# Autodesk Inventor assembly: GRIPPERFINAL51
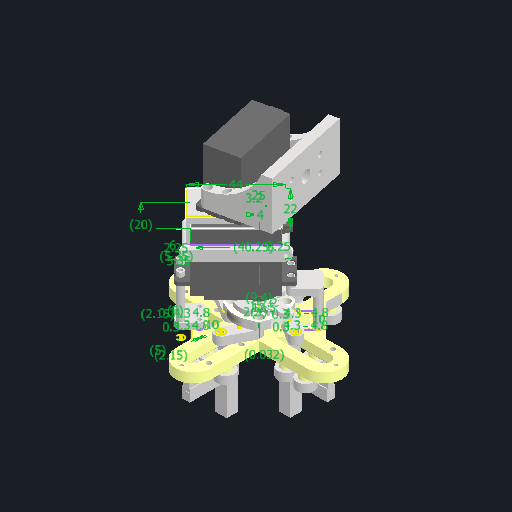
[picture p0: Inventor's stored thumbnail of the model, 512x512]
Saved by Autodesk Inventor 2026 (Build 300175000, 175)
## iProperties
Created: 2025-05-01
Part Number: GRIPPERFINAL51
Document SubType Name: Assembly
Designer: m_kni
Author: m_kni
## Documents named in this file (11)
- C:\Users\jerem\Documents\GitHub\Perovskite-Automated-Synthesis-System\CAD\Gripper\GRIPPERFINAL51.iam
- C:\Users\jerem\Documents\GitHub\Perovskite-Automated-Synthesis-System\CAD\Gripper\ALUMFINGER.ipt
- C:\Users\jerem\Documents\GitHub\Perovskite-Automated-Synthesis-System\CAD\Gripper\Assembly1.iam
- C:\Users\jerem\Documents\GitHub\Perovskite-Automated-Synthesis-System\CAD\Gripper\servostrap.ipt
- C:\Users\jerem\Documents\GitHub\Perovskite-Automated-Synthesis-System\CAD\Gripper\UpperGripperfingerpart.ipt
- C:\Users\jerem\Documents\GitHub\Perovskite-Automated-Synthesis-System\CAD\Non 3D Printed Parts\Bearings\5x5x11bearing.ipt
- C:\Users\jerem\Documents\GitHub\Perovskite-Automated-Synthesis-System\CAD\Gripper\Redesign_Linkage.ipt
- C:\Users\jerem\Documents\GitHub\Perovskite-Automated-Synthesis-System\CAD\Gripper\3x5x5bushing.ipt
- C:\Users\jerem\Documents\GitHub\Perovskite-Automated-Synthesis-System\CAD\Non 3D Printed Parts\Motors and Servos\MG 996R.ipt
- C:\Users\jerem\Documents\GitHub\Perovskite-Automated-Synthesis-System\CAD\Non 3D Printed Parts\Motors and Servos\MG996 2 Arm Pad.ipt
- C:\Users\jerem\Documents\GitHub\Perovskite-Automated-Synthesis-System\CAD\Gripper\SERVO_TO_TOOLHEAD.ipt
## Components (33 placed, 10 different names)
1. ALUMFINGER:1 — Insert:26, Angle:1
2. Assembly1:1 [sub-assembly] — Insert:1, Insert:2, Insert:3, Insert:4, Insert:5, Insert:6, Insert:7, Insert:8, Insert:9, Insert:10, Insert:11, Insert:12, Insert:13, Mate:8, Angle:5, Mate:13
3. servostrap:1 — Insert:1
4. UpperGripperfingerpart:1 — Mate:5, Tangent:3, Mate:6, Insert:29, Angle:4
5. UpperGripperfingerpart:2 — Mate:6, Tangent:4, Mate:7, Insert:27, Angle:2
6. UpperGripperfingerpart:3 — Tangent:1, Mate:1, Mate:2, Insert:28, Angle:3
7. UpperGripperfingerpart:4 — Mate:2, Tangent:2, Mate:3, Insert:26, Angle:1
8. 5x5x11bearing:1 — Insert:7
9. 5x5x11bearing:2 — Insert:6
10. 5x5x11bearing:3 — Insert:5, Tangent:1, Mate:1
11. 5x5x11bearing:4 — Insert:3, Mate:5
12. 5x5x11bearing:5 — Insert:2
13. 5x5x11bearing:6 — Insert:4, Tangent:3
14. 5x5x11bearing:7 — Insert:10, Tangent:2
15. 5x5x11bearing:8 — Insert:8
16. 5x5x11bearing:9 — Insert:11, Tangent:4, Mate:7
17. 5x5x11bearing:10 — Insert:9, Mate:3
18. 5x5x11bearing:11 — Insert:12
19. 5x5x11bearing:12 — Insert:13
20. Redesign_Linkage:1 — Insert:15
21. Redesign_Linkage:2 — Insert:24
22. Redesign_Linkage:3 — Insert:22
23. Redesign_Linkage:4 — Insert:20
24. 3x5x5bushing:5 — Insert:15
25. 3x5x5bushing:6 — Insert:22
26. 3x5x5bushing:7 — Insert:24
27. 3x5x5bushing:8 — Insert:20
28. ALUMFINGER:2 — Insert:27, Angle:2
29. ALUMFINGER:3 — Insert:28, Angle:3
30. ALUMFINGER:4 — Insert:29, Angle:4
31. MG 996R:1 — Mate:9, Mate:10, Mate:11, Mate:12, Angle:6
32. MG996 2 Arm Pad:1 — Mate:8, Angle:5, Mate:9, Mate:10, Mate:13
33. SERVO_TO_TOOLHEAD:1 — Mate:11, Mate:12, Angle:6
## Relationships (43: Insert 21, Mate 12, Angle 6, Tangent 4)
- Insert:1: Assembly1:1 ↔ servostrap:1
- Insert:2: Assembly1:1 ↔ 5x5x11bearing:5
- Insert:3: Assembly1:1 ↔ 5x5x11bearing:4
- Insert:4: Assembly1:1 ↔ 5x5x11bearing:6
- Insert:5: Assembly1:1 ↔ 5x5x11bearing:3
- Insert:6: Assembly1:1 ↔ 5x5x11bearing:2
- Insert:7: Assembly1:1 ↔ 5x5x11bearing:1
- Insert:8: Assembly1:1 ↔ 5x5x11bearing:8
- Insert:9: Assembly1:1 ↔ 5x5x11bearing:10
- Insert:10: Assembly1:1 ↔ 5x5x11bearing:7
- Insert:11: Assembly1:1 ↔ 5x5x11bearing:9
- Insert:12: Assembly1:1 ↔ 5x5x11bearing:11
- Insert:13: Assembly1:1 ↔ 5x5x11bearing:12
- Tangent:1: UpperGripperfingerpart:3 ↔ 5x5x11bearing:3
- Mate:1: UpperGripperfingerpart:3 ↔ 5x5x11bearing:3
- Insert:15: Redesign_Linkage:1 ↔ 3x5x5bushing:5
- Mate:2 (36.068 mm): UpperGripperfingerpart:3 ↔ UpperGripperfingerpart:4
- Tangent:2: UpperGripperfingerpart:4 ↔ 5x5x11bearing:7
- Mate:3: UpperGripperfingerpart:4 ↔ 5x5x11bearing:10
- Mate:5: UpperGripperfingerpart:1 ↔ 5x5x11bearing:4
- Tangent:3: UpperGripperfingerpart:1 ↔ 5x5x11bearing:6
- Mate:6 (36.068 mm): UpperGripperfingerpart:1 ↔ UpperGripperfingerpart:2
- Tangent:4: UpperGripperfingerpart:2 ↔ 5x5x11bearing:9
- Mate:7: UpperGripperfingerpart:2 ↔ 5x5x11bearing:9
- Insert:20: Redesign_Linkage:4 ↔ 3x5x5bushing:8
- Insert:22: Redesign_Linkage:3 ↔ 3x5x5bushing:6
- Insert:24: Redesign_Linkage:2 ↔ 3x5x5bushing:7
- Insert:26: ALUMFINGER:1 ↔ UpperGripperfingerpart:4
- Angle:1 (0 deg): ALUMFINGER:1 ↔ UpperGripperfingerpart:4
- Insert:27: UpperGripperfingerpart:2 ↔ ALUMFINGER:2
- Angle:2 (0 deg): UpperGripperfingerpart:2 ↔ ALUMFINGER:2
- Insert:28: UpperGripperfingerpart:3 ↔ ALUMFINGER:3
- Angle:3 (0 deg): UpperGripperfingerpart:3 ↔ ALUMFINGER:3
- Insert:29: UpperGripperfingerpart:1 ↔ ALUMFINGER:4
- Angle:4 (0 deg): UpperGripperfingerpart:1 ↔ ALUMFINGER:4
- Mate:8: Assembly1:1 ↔ MG996 2 Arm Pad:1
- Angle:5 (-9 deg): Assembly1:1 ↔ MG996 2 Arm Pad:1
- Mate:9: MG 996R:1 ↔ MG996 2 Arm Pad:1
- Mate:10: MG 996R:1 ↔ MG996 2 Arm Pad:1
- Mate:11: MG 996R:1 ↔ SERVO_TO_TOOLHEAD:1
- Mate:12: MG 996R:1 ↔ SERVO_TO_TOOLHEAD:1
- Angle:6 (0 deg): MG 996R:1 ↔ SERVO_TO_TOOLHEAD:1
- Mate:13: Assembly1:1 ↔ MG996 2 Arm Pad:1
